# Autodesk Inventor assembly: STARduino and Pi assembly
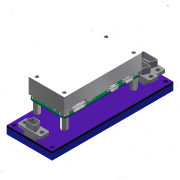
[picture p0: Inventor's stored thumbnail of the model, 180x180]
Saved by Autodesk Inventor 2017 (Build 210142000, 142)
## iProperties
Created: 2017-01-16
Part Number: STARduino and Pi assembly
Document SubType Name: Assembly
Designer: qupec
Mass: 94.0986 g
Surface Area: 327.317 cm^2
Volume: 52.2385 cm^3
Density: 1.80133 g/cm^3
Author: qupec
## Documents named in this file (12)
- D:\UMD Near Space\STAR\CAD\Mechanical\Electonics\STARduino and Pi assembly.iam
- D:\UMD Near Space\STAR\CAD\Mechanical\Electonics\STARduino layout.ipt
- D:\UMD Near Space\STAR\CAD\Mechanical\Electonics\STARduino Mount.ipt
- D:\UMD Near Space\STAR\CAD\Mechanical\Subsystems\Pi Cam\RapberryPiZero.ipt
- D:\UMD Near Space\STAR\CAD\Mechanical\Electonics\95947A005_ALUM FEM THRDED HEX STANDOFF.ipt
- D:\UMD Near Space\STAR\CAD\Mechanical\Electonics\Heat Block for Pi.ipt
- D:\UMD Near Space\STAR\CAD\Mechanical\Electonics\31pin female connector.ipt
- D:\UMD Near Space\STAR\CAD\Mechanical\Electonics\15pin female connector.ipt
- D:\UMD Near Space\STAR\CAD\Mechanical\Electonics\9pin female connector.ipt
- C:\Users\qupec\Desktop\UMD Near Space\STAR\CAD\Mechanical\31pin male connector.ipt
- C:\Users\qupec\Desktop\UMD Near Space\STAR\CAD\Mechanical\15pin male connector.ipt
- C:\Users\qupec\Desktop\UMD Near Space\STAR\CAD\Mechanical\9pin male connector.ipt
## Components (14 placed, 11 different names)
1. STARduino layout:1 — Mate:7, Mate:12, Mate:13, Mate:14, Mate:15, Mate:16, Mate:17, Mate:18, Mate:19, Mate:23, Mate:24, Mate:32, Mate:33, Mate:34, Flush:1, Flush:3, Flush:4, Flush:5, Flush:6, Flush:7
2. STARduino Mount:1 — Mate:7, Mate:23, Mate:24, Mate:44, Mate:45, Flush:8
3. RapberryPiZero:1 — Mate:26, Mate:27, Mate:28, Mate:29, Mate:30, Mate:31
4. 95947A005_ALUM FEM THRDED HEX STANDOFF:1 — Mate:13, Mate:17
5. 95947A005_ALUM FEM THRDED HEX STANDOFF:2 — Mate:12, Mate:18, Mate:29
6. 95947A005_ALUM FEM THRDED HEX STANDOFF:3 — Mate:15, Mate:16, Mate:30
7. 95947A005_ALUM FEM THRDED HEX STANDOFF:4 — Mate:14, Mate:19, Mate:31
8. Heat Block for Pi:1 — Mate:26, Mate:27, Mate:28
9. 31pin female connector:1 — Mate:34, Flush:3, Flush:5, Mate:35, Mate:40, Mate:41
10. 15pin female connector:1 — Mate:33, Mate:36, Mate:39, Mate:42, Flush:6, Flush:7
11. 9pin female connector:1 — Mate:32, Flush:1, Flush:4, Mate:37, Mate:38, Mate:43
12. 31pin male connector:1 — Mate:35, Mate:40, Mate:41
13. 15pin male connector:1 — Mate:36, Mate:39, Mate:42
14. 9pin male connector:1 — Mate:37, Mate:38, Mate:43
## Relationships (38: Mate 31, Flush 7)
- Mate:7: STARduino layout:1 ↔ STARduino Mount:1
- Mate:12: STARduino layout:1 ↔ 95947A005_ALUM FEM THRDED HEX STANDOFF:2
- Mate:13: STARduino layout:1 ↔ 95947A005_ALUM FEM THRDED HEX STANDOFF:1
- Mate:14: STARduino layout:1 ↔ 95947A005_ALUM FEM THRDED HEX STANDOFF:4
- Mate:15: STARduino layout:1 ↔ 95947A005_ALUM FEM THRDED HEX STANDOFF:3
- Mate:16: STARduino layout:1 ↔ 95947A005_ALUM FEM THRDED HEX STANDOFF:3
- Mate:17: STARduino layout:1 ↔ 95947A005_ALUM FEM THRDED HEX STANDOFF:1
- Mate:18: STARduino layout:1 ↔ 95947A005_ALUM FEM THRDED HEX STANDOFF:2
- Mate:19: STARduino layout:1 ↔ 95947A005_ALUM FEM THRDED HEX STANDOFF:4
- Mate:23: STARduino layout:1 ↔ STARduino Mount:1
- Mate:24: STARduino layout:1 ↔ STARduino Mount:1
- Mate:26: RapberryPiZero:1 ↔ Heat Block for Pi:1
- Mate:27: RapberryPiZero:1 ↔ Heat Block for Pi:1
- Mate:28: RapberryPiZero:1 ↔ Heat Block for Pi:1
- Mate:29: RapberryPiZero:1 ↔ 95947A005_ALUM FEM THRDED HEX STANDOFF:2
- Mate:30: RapberryPiZero:1 ↔ 95947A005_ALUM FEM THRDED HEX STANDOFF:3
- Mate:31: RapberryPiZero:1 ↔ 95947A005_ALUM FEM THRDED HEX STANDOFF:4
- Mate:32: STARduino layout:1 ↔ 9pin female connector:1
- Mate:33: STARduino layout:1 ↔ 15pin female connector:1
- Mate:34: STARduino layout:1 ↔ 31pin female connector:1
- Flush:1: STARduino layout:1 ↔ 9pin female connector:1
- Flush:3 (7.62 mm): STARduino layout:1 ↔ 31pin female connector:1
- Flush:4 (8.89 mm): STARduino layout:1 ↔ 9pin female connector:1
- Flush:5: STARduino layout:1 ↔ 31pin female connector:1
- Mate:35: 31pin female connector:1 ↔ 31pin male connector:1
- Mate:36: 15pin female connector:1 ↔ 15pin male connector:1
- Mate:37: 9pin female connector:1 ↔ 9pin male connector:1
- Mate:38: 9pin female connector:1 ↔ 9pin male connector:1
- Mate:39: 15pin female connector:1 ↔ 15pin male connector:1
- Mate:40: 31pin female connector:1 ↔ 31pin male connector:1
- Mate:41: 31pin female connector:1 ↔ 31pin male connector:1
- Mate:42: 15pin female connector:1 ↔ 15pin male connector:1
- Mate:43: 9pin female connector:1 ↔ 9pin male connector:1
- Flush:6: STARduino layout:1 ↔ 15pin female connector:1
- Flush:7 (6.35 mm): STARduino layout:1 ↔ 15pin female connector:1
- Mate:44: STARduino Mount:1
- Mate:45: STARduino Mount:1
- Flush:8: STARduino Mount:1
